# Autodesk Inventor assembly: клешня сбока
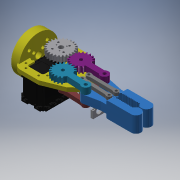
[picture p0: Inventor's stored thumbnail of the model, 180x180]
Saved by Autodesk Inventor 2019 (Build 230136000, 136)
## iProperties
Created: 2019-08-18
Part Number: клешня сбока
Material: Типовые
Document SubType Name: Assembly
Designer: Петров Иван
Mass: 103.83 g
Surface Area: 471.759 cm^2
Volume: 98.2815 cm^3
Density: 1.05645 g/cm^3
Author: Петров Иван
## Documents named in this file (11)
- E:\IVAN\Ivan_desktop\Kvantorium\Projects\optimal_gripper\hardware\КВ33.044.200 - Сборка зажима.iam
- E:\IVAN\Ivan_desktop\Kvantorium\Projects\optimal_gripper\hardware\КВ33.044.201 - Опора зажимного механизма.ipt
- E:\IVAN\Ivan_desktop\Kvantorium\Projects\optimal_gripper\hardware\КВ33.044.202 -Прихват.ipt
- E:\IVAN\Ivan_desktop\Kvantorium\Projects\optimal_gripper\hardware\КВ33.044.205 - Рычаг приводной 17 зубьев.ipt
- E:\IVAN\Ivan_desktop\Kvantorium\Projects\optimal_gripper\hardware\КВ33.044.206 - Рычаг приводной 16 зубьев.ipt
- E:\IVAN\Ivan_desktop\Kvantorium\Projects\optimal_gripper\hardware\КВ33.044.204 -Рычаг тонкий.ipt
- E:\IVAN\Ivan_desktop\Kvantorium\Projects\optimal_gripper\hardware\КВ33.044.203 - Рычаг толстый.ipt
- E:\IVAN\Ivan_desktop\Kvantorium\Projects\optimal_gripper\hardware\Стандартные изделия\Сервомотор Dynamixel AX-12A\AX-12.iam
- E:\IVAN\Ivan_desktop\Kvantorium\Projects\optimal_gripper\hardware\КВ33.044.102 - Колесо зубчатое сервомотора.ipt
- E:\IVAN\Ivan_desktop\Kvantorium\Projects\optimal_gripper\hardware\КВ33.044.207 - Крепление вакумной присоски.ipt
- E:\IVAN\Ivan_desktop\Kvantorium\Projects\optimal_gripper\hardware\КВ33.044.208 - Зажим вакумной присоски.ipt
## Components (15 placed, 10 different names)
1. КВ33.044.201 - Опора зажимного механизма:1 — Совмещение:11, Совмещение:14, Совмещение:17, Совмещение:18, Совмещение:19, Совмещение:21, Совмещение:23, Совмещение:24, Совмещение:25, Совмещение:34, Совмещение:35, Совмещение:37, Совмещение:38, Совмещение:40, Совмещение:42, Угол:1, Совмещение:50
2. КВ33.044.202 -Прихват:1 — Совмещение:12, Совмещение:13, Совмещение:15, Совмещение:16, Совмещение:26, Совмещение:33, Совмещение:36
3. КВ33.044.202 -Прихват:2 — Совмещение:9, Совмещение:10, Совмещение:20, Совмещение:22, Совмещение:32, Совмещение:39
4. КВ33.044.204 -Рычаг тонкий:1 — Совмещение:9, Совмещение:10, Совмещение:11, Совмещение:46
5. КВ33.044.204 -Рычаг тонкий:2 — Совмещение:12, Совмещение:13, Совмещение:14, Совмещение:45
6. КВ33.044.204 -Рычаг тонкий:3 — Совмещение:15, Совмещение:16, Совмещение:17
7. КВ33.044.204 -Рычаг тонкий:4 — Совмещение:18, Совмещение:19, Совмещение:20
8. КВ33.044.203 - Рычаг толстый:1 — Совмещение:24, Совмещение:25, Совмещение:26, Совмещение:33
9. КВ33.044.203 - Рычаг толстый:2 — Совмещение:21, Совмещение:22, Совмещение:23, Совмещение:32
10. AX-12:1 [sub-assembly] — Совмещение:40, Совмещение:42, Совмещение:43, Совмещение:44, Совмещение:50
11. КВ33.044.102 - Колесо зубчатое сервомотора:1 — Направление навивки:1, Совмещение:43, Совмещение:44
12. КВ33.044.205 - Рычаг приводной 17 зубьев:1 — Совмещение:34, Совмещение:35, Совмещение:36, Направление навивки:1, Направление навивки:2
13. КВ33.044.206 - Рычаг приводной 16 зубьев:1 — Совмещение:37, Совмещение:38, Совмещение:39, Направление навивки:2
14. КВ33.044.207 - Крепление вакумной присоски:1 — Совмещение:45, Совмещение:46, Угол:1, Совмещение:47, Совмещение:48, Совмещение:49
15. КВ33.044.208 - Зажим вакумной присоски:1 — Совмещение:47, Совмещение:48, Совмещение:49
## Relationships (39: Mate 36, RelateRotation 2, Angle 1)
- Совмещение:9 [Mate]: КВ33.044.202 -Прихват:2 ↔ КВ33.044.204 -Рычаг тонкий:1
- Совмещение:10 [Mate]: КВ33.044.202 -Прихват:2 ↔ КВ33.044.204 -Рычаг тонкий:1
- Совмещение:11 [Mate]: КВ33.044.201 - Опора зажимного механизма:1 ↔ КВ33.044.204 -Рычаг тонкий:1
- Совмещение:12 [Mate]: КВ33.044.202 -Прихват:1 ↔ КВ33.044.204 -Рычаг тонкий:2
- Совмещение:13 [Mate]: КВ33.044.202 -Прихват:1 ↔ КВ33.044.204 -Рычаг тонкий:2
- Совмещение:14 [Mate]: КВ33.044.201 - Опора зажимного механизма:1 ↔ КВ33.044.204 -Рычаг тонкий:2
- Совмещение:15 [Mate]: КВ33.044.202 -Прихват:1 ↔ КВ33.044.204 -Рычаг тонкий:3
- Совмещение:16 [Mate]: КВ33.044.202 -Прихват:1 ↔ КВ33.044.204 -Рычаг тонкий:3
- Совмещение:17 [Mate]: КВ33.044.201 - Опора зажимного механизма:1 ↔ КВ33.044.204 -Рычаг тонкий:3
- Совмещение:18 [Mate]: КВ33.044.201 - Опора зажимного механизма:1 ↔ КВ33.044.204 -Рычаг тонкий:4
- Совмещение:19 [Mate]: КВ33.044.201 - Опора зажимного механизма:1 ↔ КВ33.044.204 -Рычаг тонкий:4
- Совмещение:20 [Mate]: КВ33.044.202 -Прихват:2 ↔ КВ33.044.204 -Рычаг тонкий:4
- Совмещение:21 [Mate]: КВ33.044.201 - Опора зажимного механизма:1 ↔ КВ33.044.203 - Рычаг толстый:2
- Совмещение:22 [Mate]: КВ33.044.202 -Прихват:2 ↔ КВ33.044.203 - Рычаг толстый:2
- Совмещение:23 [Mate]: КВ33.044.201 - Опора зажимного механизма:1 ↔ КВ33.044.203 - Рычаг толстый:2
- Совмещение:24 [Mate]: КВ33.044.201 - Опора зажимного механизма:1 ↔ КВ33.044.203 - Рычаг толстый:1
- Совмещение:25 [Mate]: КВ33.044.201 - Опора зажимного механизма:1 ↔ КВ33.044.203 - Рычаг толстый:1
- Совмещение:26 [Mate]: КВ33.044.202 -Прихват:1 ↔ КВ33.044.203 - Рычаг толстый:1
- Совмещение:32 [Mate]: КВ33.044.202 -Прихват:2 ↔ КВ33.044.203 - Рычаг толстый:2
- Совмещение:33 [Mate]: КВ33.044.202 -Прихват:1 ↔ КВ33.044.203 - Рычаг толстый:1
- Совмещение:34 [Mate]: КВ33.044.201 - Опора зажимного механизма:1 ↔ КВ33.044.205 - Рычаг приводной 17 зубьев:1
- Совмещение:35 [Mate]: КВ33.044.201 - Опора зажимного механизма:1 ↔ КВ33.044.205 - Рычаг приводной 17 зубьев:1
- Совмещение:36 [Mate]: КВ33.044.202 -Прихват:1 ↔ КВ33.044.205 - Рычаг приводной 17 зубьев:1
- Совмещение:37 [Mate]: КВ33.044.201 - Опора зажимного механизма:1 ↔ КВ33.044.206 - Рычаг приводной 16 зубьев:1
- Совмещение:38 [Mate]: КВ33.044.201 - Опора зажимного механизма:1 ↔ КВ33.044.206 - Рычаг приводной 16 зубьев:1
- Совмещение:39 [Mate]: КВ33.044.202 -Прихват:2 ↔ КВ33.044.206 - Рычаг приводной 16 зубьев:1
- Направление навивки:1 [RelateRotation] (1.5 ul): КВ33.044.102 - Колесо зубчатое сервомотора:1 ↔ КВ33.044.205 - Рычаг приводной 17 зубьев:1
- Направление навивки:2 [RelateRotation] (1 ul): КВ33.044.205 - Рычаг приводной 17 зубьев:1 ↔ КВ33.044.206 - Рычаг приводной 16 зубьев:1
- Совмещение:40 [Mate]: КВ33.044.201 - Опора зажимного механизма:1 ↔ AX-12:1
- Совмещение:42 [Mate]: КВ33.044.201 - Опора зажимного механизма:1 ↔ AX-12:1
- Совмещение:43 [Mate]: AX-12:1 ↔ КВ33.044.102 - Колесо зубчатое сервомотора:1
- Совмещение:44 [Mate]: AX-12:1 ↔ КВ33.044.102 - Колесо зубчатое сервомотора:1
- Совмещение:45 [Mate]: КВ33.044.204 -Рычаг тонкий:2 ↔ КВ33.044.207 - Крепление вакумной присоски:1
- Совмещение:46 [Mate]: КВ33.044.204 -Рычаг тонкий:1 ↔ КВ33.044.207 - Крепление вакумной присоски:1
- Угол:1 [Angle] (0 deg): КВ33.044.201 - Опора зажимного механизма:1 ↔ КВ33.044.207 - Крепление вакумной присоски:1
- Совмещение:47 [Mate]: КВ33.044.207 - Крепление вакумной присоски:1 ↔ КВ33.044.208 - Зажим вакумной присоски:1
- Совмещение:48 [Mate]: КВ33.044.207 - Крепление вакумной присоски:1 ↔ КВ33.044.208 - Зажим вакумной присоски:1
- Совмещение:49 [Mate]: КВ33.044.207 - Крепление вакумной присоски:1 ↔ КВ33.044.208 - Зажим вакумной присоски:1
- Совмещение:50 [Mate]: КВ33.044.201 - Опора зажимного механизма:1 ↔ AX-12:1
